# Autodesk Inventor assembly: Assembly1
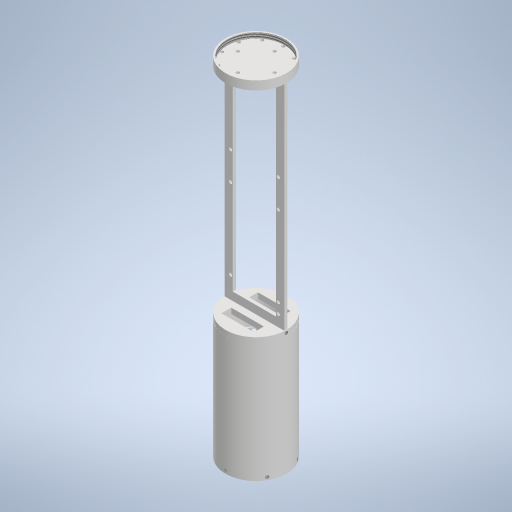
[picture p0: Inventor's stored thumbnail of the model, 512x512]
Saved by Autodesk Inventor 2023 (Build 270158000, 158)
## iProperties
Created: 2022-07-12
Part Number: Assembly1
Document SubType Name: Assembly
Designer: samlo
Author: samlo
## Documents named in this file (3)
- D:\Documents\reaction-wheel\CAD\Assembly1.iam
- D:\Documents\reaction-wheel\CAD\battery holder.ipt
- D:\Documents\reaction-wheel\CAD\case v0.ipt
## Components (2 placed, 2 different names)
1. battery holder:1 — Mate:1
2. case v0:1 — Mate:1
## Relationships (1: Mate 1)
- Mate:1: battery holder:1 ↔ case v0:1
